# Autodesk Inventor assembly: 6P Sprocket
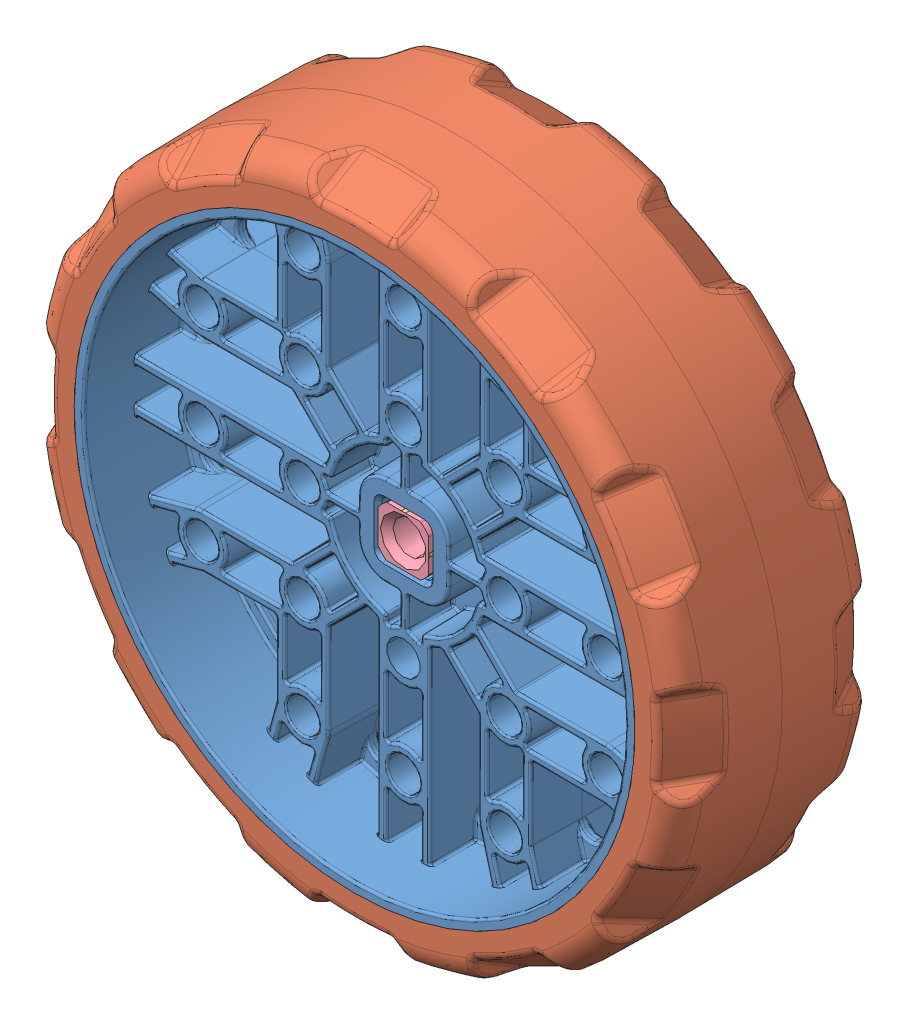
[picture p0: shaded view drawn from the shape stored in the file]
Saved by Autodesk Inventor 2026.2 (Build 302298000, 298)
## iProperties
Created: 2022-08-02
Part Number: 6P Sprocket
Document SubType Name: Assembly
Designer: ylu12
Author: ylu12
## Documents named in this file (4)
- C:\Personal\Deprecated\VEX V5 Push Back\S-bot-two\CAD\VEX-CAD-Inventor-1.4.2\Motion\Wheels\Traction Wheel\3.25 Traction AS, Circle.iam
- C:\Personal\Deprecated\VEX V5 Push Back\S-bot-two\CAD\VEX-CAD-Inventor-1.4.2\Motion\Wheels\Reference Files\3.25 Traction Antistatic.ipt
- C:\Personal\Deprecated\VEX V5 Push Back\S-bot-two\CAD\VEX-CAD-Inventor-1.4.2\Motion\HS Shaft Adapter Circle.ipt
- C:\Personal\Deprecated\VEX V5 Push Back\S-bot-two\CAD\VEX-CAD-Inventor-1.4.2\Motion\Wheels\Traction Wheel.iam
## Components (2 placed, 2 different names)
1. 3.25 Traction Antistatic:1 — Mate:20, Mate:22, Mate:24
2. Circle — Mate:32, Mate:33, Flush:10
## Relationships (6: Mate 5, Flush 1)
- Mate:20: 3.25 Traction Antistatic:1
- Mate:22: 3.25 Traction Antistatic:1
- Mate:24: 3.25 Traction Antistatic:1
- Mate:32: Circle
- Mate:33: Circle
- Flush:10 (6.35 mm): Circle
## Named parameters: Thickness = 8.255 mm
